# Autodesk Inventor assembly: pulley_case
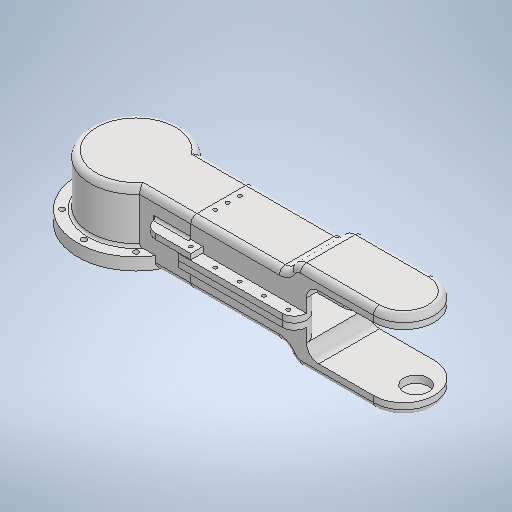
[picture p0: Inventor's stored thumbnail of the model, 512x512]
Saved by Autodesk Inventor 2025 (Build 290162000, 162)
## iProperties
Created: 2025-02-04
Part Number: pulley_case
Document SubType Name: Assembly
Designer: danielrachi
Author: danielrachi
## Documents named in this file (3)
- C:\Users\danielrachi\Documents\pulley_case.iam
- C:\Users\danielrachi\Documents\pulley_case_part_1.ipt
- C:\Users\danielrachi\Documents\pulley_case_part_2_v2.ipt
## Components (3 placed, 2 different names)
1. pulley_case_part_1:1 — Flush:1, Flush:2, Mate:1, Flush:3, Flush:4, Mate:2
2. pulley_case_part_2_v2:1 — Flush:1, Flush:2, Mate:1
3. pulley_case_part_2_v2:2 — Flush:3, Flush:4, Mate:2
## Relationships (6: Flush 4, Mate 2)
- Flush:1: pulley_case_part_1:1 ↔ pulley_case_part_2_v2:1
- Flush:2: pulley_case_part_1:1 ↔ pulley_case_part_2_v2:1
- Mate:1: pulley_case_part_1:1 ↔ pulley_case_part_2_v2:1
- Flush:3: pulley_case_part_1:1 ↔ pulley_case_part_2_v2:2
- Flush:4: pulley_case_part_1:1 ↔ pulley_case_part_2_v2:2
- Mate:2: pulley_case_part_1:1 ↔ pulley_case_part_2_v2:2
